# Autodesk Inventor assembly: ShooterAssemblyV03
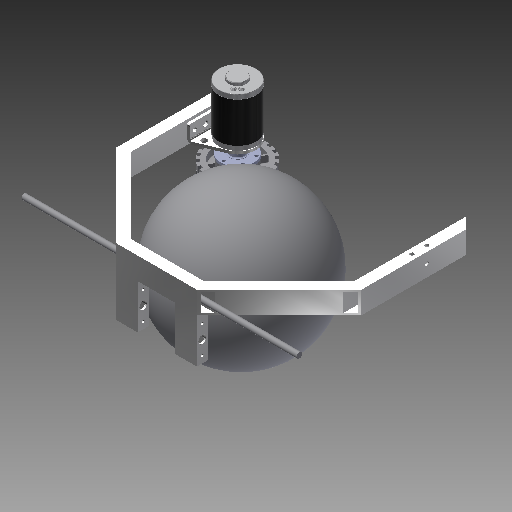
[picture p0: Inventor's stored thumbnail of the model, 512x512]
Saved by Autodesk Inventor 2017 SP1 (Build 210196100, 196)
## iProperties
Created: 2016-02-07
Part Number: ShooterAssemblyV03
Document SubType Name: Assembly
Designer: steele
Author: steele
## Documents named in this file (5)
- D:\snobotics\CAD-Development\robSteele\SnoBotics2016\2016-05-05-ShooterPrototype\ShooterAssemblyV03.iam
- D:\snobotics\CAD-Development\robSteele\SnoBotics2016\2016-05-05-ShooterPrototype\ShooterFrameV02.ipt
- D:\snobotics\CAD-Development\robSteele\SnoBotics2016\DraftOfBoulder.ipt
- D:\snobotics\CAD-Development\robSteele\SnoBotics2016\2016-05-05-ShooterPrototype\3_8_Rod.ipt
- D:\snobotics\CAD-Development\robSteele\SnoBotics2016\2016-05-05-ShooterPrototype\Mini_CIM_MotorHub_4_inch_wheel.iam
## Components (4 placed, 4 different names)
1. ShooterFrameV02:1 — Mate:1, Flush:1, Flush:2, Mate:2, Mate:4, Insert:1
2. Mini_CIM_MotorHub_4_inch_wheel:1 [sub-assembly] — Mate:1, Flush:1, Flush:2, Mate:3
3. DraftOfBoulder:1 — Mate:2, Mate:3, Mate:4
4. 3_8_Rod:1 — Insert:1
## Relationships (7: Mate 4, Flush 2, Insert 1)
- Mate:1: ShooterFrameV02:1 ↔ Mini_CIM_MotorHub_4_inch_wheel:1
- Flush:1: ShooterFrameV02:1 ↔ Mini_CIM_MotorHub_4_inch_wheel:1
- Flush:2 (-4.7625 mm): ShooterFrameV02:1 ↔ Mini_CIM_MotorHub_4_inch_wheel:1
- Mate:2: ShooterFrameV02:1 ↔ DraftOfBoulder:1
- Mate:3: Mini_CIM_MotorHub_4_inch_wheel:1 ↔ DraftOfBoulder:1
- Mate:4: ShooterFrameV02:1 ↔ DraftOfBoulder:1
- Insert:1 (25.4 mm): ShooterFrameV02:1 ↔ 3_8_Rod:1
